# Autodesk Inventor assembly: ParallelMech_Base_V2_Assembly
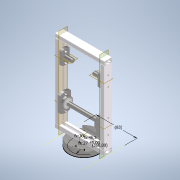
[picture p0: Inventor's stored thumbnail of the model, 180x180]
Saved by Autodesk Inventor 2022 (Build 260153000, 153)
## iProperties
Created: 2022-08-03
Part Number: ParallelMech_Base_V2_Assembly
Document SubType Name: Assembly
Designer: alexw
LinkDist_ParallelMecha: 80,000 mm
BaseFrame_InnerWidth: 83,000 mm
Author: alexw
## Documents named in this file (4)
- C:\Users\alexw\Documents\Inventor\Projects\03_CurrentProjects\MasterThesis\PSM_V1_Rillenkugellager\ParallelMech_Base_V2_Assembly.iam
- C:\Users\alexw\Documents\Inventor\Projects\03_CurrentProjects\MasterThesis\PSM_V1_Rillenkugellager\Flansch_FemalePart_MainAxis_HeadConnectorBase_V2.ipt
- C:\Users\alexw\Documents\Inventor\Projects\03_CurrentProjects\MasterThesis\PSM_V1_Rillenkugellager\ParallelMecha_V2_BaseFrame_Item.iam
- C:\Users\alexw\Documents\Inventor\Projects\03_CurrentProjects\MasterThesis\PSM_V1_Rillenkugellager\ContentCenter\de-DE\ISO 10642(1)\ISO 10642 - M4 x  12.ipt
## Components (4 placed, 3 different names)
1. Flansch_FemalePart_MainAxis_HeadConnectorBase_V2:1 — Passend:7, Passend:8, Fluchtend:3, Fluchtend:4, Fluchtend:5, Passend:9
2. ParallelMecha_V2_BaseFrame_Item:1 [sub-assembly] — Passend:9, Passend:10, Passend:11
3. ISO 10642 M4x12:1 — Passend:7, Passend:10
4. ISO 10642 M4x12:2 — Passend:8, Passend:11
## Relationships (8: Mate 5, Flush 3)
- Passend:7 [Mate]: Flansch_FemalePart_MainAxis_HeadConnectorBase_V2:1 ↔ ISO 10642 M4x12:1
- Passend:8 [Mate]: Flansch_FemalePart_MainAxis_HeadConnectorBase_V2:1 ↔ ISO 10642 M4x12:2
- Fluchtend:3 [Flush]: Flansch_FemalePart_MainAxis_HeadConnectorBase_V2:1
- Fluchtend:4 [Flush]: Flansch_FemalePart_MainAxis_HeadConnectorBase_V2:1
- Fluchtend:5 [Flush]: Flansch_FemalePart_MainAxis_HeadConnectorBase_V2:1
- Passend:9 [Mate]: Flansch_FemalePart_MainAxis_HeadConnectorBase_V2:1 ↔ ParallelMecha_V2_BaseFrame_Item:1
- Passend:10 [Mate]: ParallelMecha_V2_BaseFrame_Item:1 ↔ ISO 10642 M4x12:1
- Passend:11 [Mate]: ParallelMecha_V2_BaseFrame_Item:1 ↔ ISO 10642 M4x12:2
## Named parameters: LinkDist_ParallelMecha = 80 mm, ProximalOffset2Base_LinkFixation_Proximal = 30 mm, BaseFrame_InnerWidth = 83 mm
